# Autodesk Inventor assembly: Gantry_LaserHolder
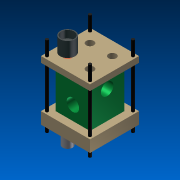
[picture p0: Inventor's stored thumbnail of the model, 180x180]
Saved by Autodesk Inventor 2012 (Build 160160000, 160)
## iProperties
Created: 2012-03-02
Part Number: Gantry_LaserHolder
Document SubType Name: Assembly
Designer: German
Author: German
## Documents named in this file (3)
- C:\Users\German\Desktop\Laser_Etching\Gantry_LaserHolder.iam
- C:\Users\German\Desktop\Laser_Etching\LaserHolder.iam
- C:\Users\German\Desktop\Laser_Etching\basicgantry.iam
## Components (2 placed, 2 different names)
1. LaserHolder:1 [sub-assembly] — Insert:1
2. basicgantry:1 [sub-assembly] — Insert:1
## Relationships (1: Insert 1)
- Insert:1 (-11 mm): LaserHolder:1 ↔ basicgantry:1
